# Autodesk Inventor assembly: Whistle Mk 2.1
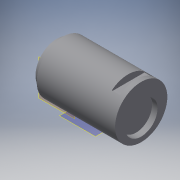
[picture p0: Inventor's stored thumbnail of the model, 180x180]
Saved by Autodesk Inventor 2019 (Build 230136000, 136)
## iProperties
Created: 2019-04-01
Part Number: Whistle Mk 2.1
Document SubType Name: Assembly
Designer: Kepler
Author: Kepler
## Documents named in this file (4)
- C:\Users\Kepler\Documents\Inventor\Whistles\Whistle Mk 2.1.iam
- C:\Users\Kepler\Documents\Inventor\Whistles\Whistle Exterior 2.1.ipt
- C:\Users\Kepler\Documents\Inventor\Whistles\Whistle 1.2.ipt
- C:\Users\Kepler\Documents\Inventor\Whistles\Air Restricter 1.ipt
## Components (3 placed, 3 different names)
1. Whistle Exterior 2.1:1 — Mate:1, Flush:1, Mate:2, Mate:3
2. Whistle 1.2:1 — Mate:1, Flush:1
3. Air Restricter 1:1 — Mate:2, Mate:3
## Relationships (4: Mate 3, Flush 1)
- Mate:1: Whistle Exterior 2.1:1 ↔ Whistle 1.2:1
- Flush:1: Whistle Exterior 2.1:1 ↔ Whistle 1.2:1
- Mate:2 (0.25 mm): Whistle Exterior 2.1:1 ↔ Air Restricter 1:1
- Mate:3 (0.25 mm): Whistle Exterior 2.1:1 ↔ Air Restricter 1:1
